# Autodesk Inventor assembly: 15102898-16-A-0800
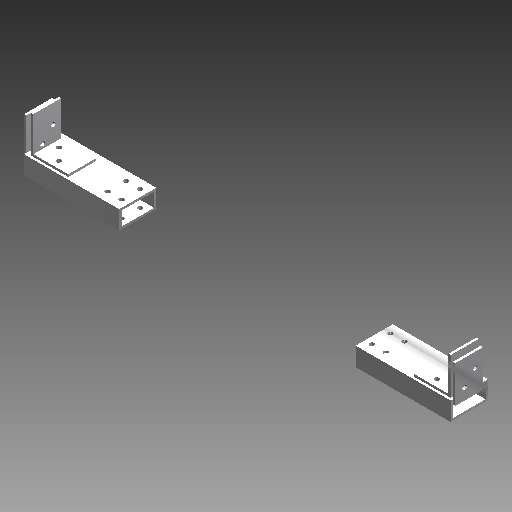
[picture p0: Inventor's stored thumbnail of the model, 512x512]
Saved by Autodesk Inventor 2017 (Build 210142000, 142)
## iProperties
Created: 2016-10-10
Part Number: 15102898-16-A-0800
Document SubType Name: Assembly
Designer: gus
Mass: 429.517 g
Surface Area: 1079.84 cm^2
Volume: 159.081 cm^3
Density: 2.7 g/cm^3
Author: gus
## Documents named in this file (6)
- \\Mac\Home\Desktop\bunnybots 2016\15102898-16-Bunnybot-CAD\Bunnybot-Night_Fury\15102898-16-A-0000\15102898-16-A-0800\15102898-16-A-0800.iam
- \\Mac\Home\Desktop\bunnybots 2016\15102898-16-Bunnybot-CAD\Bunnybot-Night_Fury\15102898-16-A-0000\15102898-16-A-0800\15102898-16-P-0801.ipt
- \\Mac\Home\Desktop\bunnybots 2016\15102898-16-Bunnybot-CAD\Bunnybot-Night_Fury\15102898-16-A-0000\15102898-16-A-0800\15102898-16-P-0802.ipt
- \\Mac\Home\Desktop\bunnybots 2016\15102898-16-Bunnybot-CAD\Bunnybot-Night_Fury\15102898-16-A-0000\15102898-16-A-0800\15102898-16-P-0803.ipt
- \\Mac\Home\Desktop\bunnybots 2016\15102898-16-Bunnybot-CAD\Bunnybot-Night_Fury\15102898-16-A-0000\15102898-16-A-0800\15102898-16-P-0804.ipt
- \\Mac\Home\Desktop\bunnybots 2016\15102898-16-Bunnybot-CAD\Bunnybot-Night_Fury\15102898-16-A-0000\15102898-16-A-0800\15102898-16-P-0805.ipt
## Components (6 placed, 5 different names)
1. 15102898-16-P-0801:1 — Flush:1, Flush:2, Mate:1, Mate:2, Mate:3, Mate:4, Mate:8
2. 15102898-16-P-0801:2 — Flush:1, Flush:2, Mate:1, Mate:5, Mate:6, Mate:7, Mate:10
3. 15102898-16-P-0802:1 — Mate:2, Mate:3, Mate:4, Flush:3, Mate:9
4. 15102898-16-P-0803:1 — Mate:5, Mate:6, Mate:7, Mate:11, Flush:4
5. 15102898-16-P-0804:1 — Mate:8, Flush:3, Mate:9
6. 15102898-16-P-0805:1 — Mate:10, Mate:11, Flush:4
## Relationships (15: Mate 11, Flush 4)
- Flush:1: 15102898-16-P-0801:1 ↔ 15102898-16-P-0801:2
- Flush:2: 15102898-16-P-0801:1 ↔ 15102898-16-P-0801:2
- Mate:1 (323.596 mm): 15102898-16-P-0801:1 ↔ 15102898-16-P-0801:2
- Mate:2: 15102898-16-P-0801:1 ↔ 15102898-16-P-0802:1
- Mate:3: 15102898-16-P-0801:1 ↔ 15102898-16-P-0802:1
- Mate:4: 15102898-16-P-0801:1 ↔ 15102898-16-P-0802:1
- Mate:5: 15102898-16-P-0801:2 ↔ 15102898-16-P-0803:1
- Mate:6: 15102898-16-P-0801:2 ↔ 15102898-16-P-0803:1
- Mate:7: 15102898-16-P-0801:2 ↔ 15102898-16-P-0803:1
- Mate:8: 15102898-16-P-0801:1 ↔ 15102898-16-P-0804:1
- Flush:3: 15102898-16-P-0802:1 ↔ 15102898-16-P-0804:1
- Mate:9 (3.175 mm): 15102898-16-P-0802:1 ↔ 15102898-16-P-0804:1
- Mate:10: 15102898-16-P-0801:2 ↔ 15102898-16-P-0805:1
- Mate:11 (6.35 mm): 15102898-16-P-0803:1 ↔ 15102898-16-P-0805:1
- Flush:4: 15102898-16-P-0803:1 ↔ 15102898-16-P-0805:1
